# Autodesk Inventor assembly: Podstawa+Kola+Obudowa
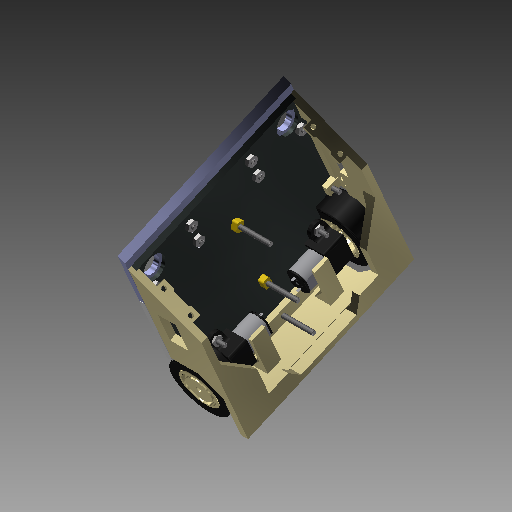
[picture p0: Inventor's stored thumbnail of the model, 512x512]
Saved by Autodesk Inventor 2017 (Build 210142000, 142)
## iProperties
Created: 2016-11-21
Part Number: Podstawa+Kola+Obudowa
Document SubType Name: Assembly
Designer: Shichi
Author: Shichi
## Documents named in this file (6)
- E:\h3fty\H3FTY\Model\1. Podstawa+Kola+Obudowa.iam
- E:\h3fty\H3FTY\Model\Podstawy\Podstawa_zlozona+Sruby.iam
- E:\h3fty\H3FTY\Model\Koła\Koło+Opona+Silnik.iam
- E:\h3fty\H3FTY\Model\Inne\Obudowa.ipt
- C:\Users\Shichi\Documents\Inventor\Content Center Files\R2017\en-US\AS 1112 (2)\AS 1112 - M2,5  Type 5.ipt
- E:\h3fty\H3FTY\Model\Inne\Podkladka.ipt
## Components (10 placed, 5 different names)
1. Podstawa_zlozona+Sruby:1 [sub-assembly] — Insert:1, Insert:2, Insert:3, Insert:4, Insert:5, Insert:6, Insert:11, Insert:12
2. Koło+Opona+Silnik:1 [sub-assembly] — Insert:3, Insert:4, Insert:7, Insert:8
3. Koło+Opona+Silnik:2 [sub-assembly] — Insert:1, Insert:2, Insert:9, Insert:10
4. Obudowa:1 — Insert:5, Insert:6
5. AS 1112 (2) - Metric M2,5  Type 5:1 — Insert:10
6. AS 1112 (2) - Metric M2,5  Type 5:2 — Insert:7
7. AS 1112 (2) - Metric M2,5  Type 5:4 — Insert:8
8. AS 1112 (2) - Metric M2,5  Type 5:5 — Insert:9
9. Podkladka:1 — Insert:11
10. Podkladka:2 — Insert:12
## Relationships (12: Insert 12)
- Insert:1: Podstawa_zlozona+Sruby:1 ↔ Koło+Opona+Silnik:2
- Insert:2: Podstawa_zlozona+Sruby:1 ↔ Koło+Opona+Silnik:2
- Insert:3: Podstawa_zlozona+Sruby:1 ↔ Koło+Opona+Silnik:1
- Insert:4: Podstawa_zlozona+Sruby:1 ↔ Koło+Opona+Silnik:1
- Insert:5: Podstawa_zlozona+Sruby:1 ↔ Obudowa:1
- Insert:6: Podstawa_zlozona+Sruby:1 ↔ Obudowa:1
- Insert:7: Koło+Opona+Silnik:1 ↔ AS 1112 (2) - Metric M2,5  Type 5:2
- Insert:8: Koło+Opona+Silnik:1 ↔ AS 1112 (2) - Metric M2,5  Type 5:4
- Insert:9: Koło+Opona+Silnik:2 ↔ AS 1112 (2) - Metric M2,5  Type 5:5
- Insert:10: Koło+Opona+Silnik:2 ↔ AS 1112 (2) - Metric M2,5  Type 5:1
- Insert:11: Podstawa_zlozona+Sruby:1 ↔ Podkladka:1
- Insert:12: Podstawa_zlozona+Sruby:1 ↔ Podkladka:2
